# Autodesk Inventor assembly: Case Top
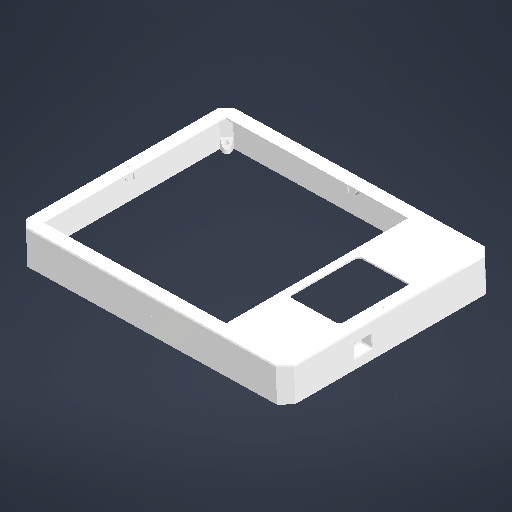
[picture p0: Inventor's stored thumbnail of the model, 512x512]
Saved by Autodesk Inventor 2026 (Build 300175000, 175)
## iProperties
Created: 2025-06-13
Part Number: Case Top
Document SubType Name: Assembly
Designer: ckyiu
Author: ckyiu
## Documents named in this file (8)
- F:\Chessboard-Design\Design\Case\Top\Case Top.iam
- F:\Chessboard-Design\Design\Case\Top\Case Top BR.ipt
- F:\Chessboard-Design\Design\Case\Top\Case Top TL.ipt
- F:\Chessboard-Design\Design\Case\Top\Case Top TR.ipt
- F:\Chessboard-Design\Design\Case\Top\Case Top BL.ipt
- F:\Chessboard-Design\Design\Hardware\M2.5\Heat set inserts\(4mm) 94459A768_Heat-Set Inserts for Plastic.ipt
- F:\Chessboard-Design\Design\Hardware\M2.5\Screws\(12mm) 92000A107_Passivated 18-8 Stainless Steel Pan Head Phillips Screws.ipt
- F:\Chessboard-Design\Design\Hardware\M2.5\Nuts\(2mm) 91828A113_18-8 Stainless Steel Hex Nut.ipt
## Components (16 placed, 7 different names)
1. Case Top BR:1 — Mate:1, Mate:4, Flush:1, Flush:2, Flush:3, Flush:4, Insert:2, Insert:5, Insert:11
2. Case Top TL:1 — Mate:2, Mate:3, Flush:5, Insert:4, Insert:7, Insert:9
3. Case Top TR:1 — Mate:3, Mate:4, Flush:1, Flush:4, Flush:5, Insert:1, Insert:8, Insert:10
4. Case Top BL:1 — Mate:1, Mate:2, Flush:2, Flush:3, Insert:3, Insert:6, Insert:12
5. (4mm) 94459A768_Heat-Set Inserts for Plastic:1 — Insert:3
6. (4mm) 94459A768_Heat-Set Inserts for Plastic:2 — Insert:4
7. (4mm) 94459A768_Heat-Set Inserts for Plastic:3 — Insert:2
8. (4mm) 94459A768_Heat-Set Inserts for Plastic:4 — Insert:1
9. (12mm) 92000A107_Passivated 18-8 Stainless Steel Pan Head Phillips Screws:1 — Insert:5
10. (12mm) 92000A107_Passivated 18-8 Stainless Steel Pan Head Phillips Screws:2 — Insert:6
11. (12mm) 92000A107_Passivated 18-8 Stainless Steel Pan Head Phillips Screws:3 — Insert:8
12. (12mm) 92000A107_Passivated 18-8 Stainless Steel Pan Head Phillips Screws:4 — Insert:7
13. (2mm) 91828A113_18-8 Stainless Steel Hex Nut:1 — Insert:9
14. (2mm) 91828A113_18-8 Stainless Steel Hex Nut:2 — Insert:12
15. (2mm) 91828A113_18-8 Stainless Steel Hex Nut:3 — Insert:11
16. (2mm) 91828A113_18-8 Stainless Steel Hex Nut:4 — Insert:10
## Relationships (21: Insert 12, Flush 5, Mate 4)
- Mate:1: Case Top BR:1 ↔ Case Top BL:1
- Mate:2: Case Top TL:1 ↔ Case Top BL:1
- Mate:3: Case Top TL:1 ↔ Case Top TR:1
- Mate:4: Case Top BR:1 ↔ Case Top TR:1
- Flush:1: Case Top BR:1 ↔ Case Top TR:1
- Flush:2: Case Top BR:1 ↔ Case Top BL:1
- Flush:3: Case Top BR:1 ↔ Case Top BL:1
- Flush:4: Case Top BR:1 ↔ Case Top TR:1
- Flush:5: Case Top TL:1 ↔ Case Top TR:1
- Insert:1 (-0.01 mm): Case Top TR:1 ↔ (4mm) 94459A768_Heat-Set Inserts for Plastic:4
- Insert:2 (-0.01 mm): Case Top BR:1 ↔ (4mm) 94459A768_Heat-Set Inserts for Plastic:3
- Insert:3 (-0.01 mm): Case Top BL:1 ↔ (4mm) 94459A768_Heat-Set Inserts for Plastic:1
- Insert:4 (-0.01 mm): Case Top TL:1 ↔ (4mm) 94459A768_Heat-Set Inserts for Plastic:2
- Insert:5: Case Top BR:1 ↔ (12mm) 92000A107_Passivated 18-8 Stainless Steel Pan Head Phillips Screws:1
- Insert:6: Case Top BL:1 ↔ (12mm) 92000A107_Passivated 18-8 Stainless Steel Pan Head Phillips Screws:2
- Insert:7: Case Top TL:1 ↔ (12mm) 92000A107_Passivated 18-8 Stainless Steel Pan Head Phillips Screws:4
- Insert:8: Case Top TR:1 ↔ (12mm) 92000A107_Passivated 18-8 Stainless Steel Pan Head Phillips Screws:3
- Insert:9: Case Top TL:1 ↔ (2mm) 91828A113_18-8 Stainless Steel Hex Nut:1
- Insert:10: Case Top TR:1 ↔ (2mm) 91828A113_18-8 Stainless Steel Hex Nut:4
- Insert:11: Case Top BR:1 ↔ (2mm) 91828A113_18-8 Stainless Steel Hex Nut:3
- Insert:12: Case Top BL:1 ↔ (2mm) 91828A113_18-8 Stainless Steel Hex Nut:2
